# Autodesk Inventor assembly: MyPart_V0_with_case
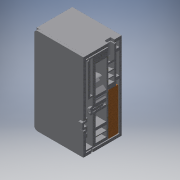
[picture p0: Inventor's stored thumbnail of the model, 180x180]
Saved by Autodesk Inventor 2016 (Build 200138000, 138)
## iProperties
Created: 2016-10-30
Part Number: MyPart_V0_with_case
Document SubType Name: Assembly
Designer: rawrdong
Author: rawrdong
## Documents named in this file (5)
- C:\Users\rawrdong\Box Sync\0_GradSchoolResearch\00_projects\0_AirParticleCounter\NEW_SHIT\MECH_E\MyPart_V0_with_case.iam
- C:\Users\rawrdong\Box Sync\0_GradSchoolResearch\00_projects\0_AirParticleCounter\NEW_SHIT\MECH_E\MyPart_V0.iam
- C:\Users\rawrdong\Box Sync\0_GradSchoolResearch\00_projects\0_AirParticleCounter\NEW_SHIT\MECH_E\case_button.ipt
- C:\Users\rawrdong\Box Sync\0_GradSchoolResearch\00_projects\0_AirParticleCounter\NEW_SHIT\MECH_E\case_carabiner.ipt
- C:\Users\rawrdong\Box Sync\0_GradSchoolResearch\00_projects\0_AirParticleCounter\NEW_SHIT\MECH_E\case_lid.ipt
## Components (4 placed, 4 different names)
1. MyPart_V0:1 [sub-assembly] — Mate:1, Flush:3, Flush:4, Flush:7, Flush:8
2. case_button:1 — Mate:3, Mate:4, Angle:1
3. case_carabiner:1 — Mate:1, Flush:1, Flush:2, Mate:2, Flush:5, Flush:6, Flush:9, Flush:10
4. case_lid:1 — Flush:1, Flush:2, Mate:2, Mate:3, Mate:4, Angle:1
## Relationships (21: Flush 10, Mate 6, Symmetry 4, Angle 1)
- Mate:1: MyPart_V0:1 ↔ case_carabiner:1
- Flush:1: case_carabiner:1 ↔ case_lid:1
- Flush:2: case_carabiner:1 ↔ case_lid:1
- Mate:2: case_carabiner:1 ↔ case_lid:1
- Mate:3: case_button:1 ↔ case_lid:1
- Mate:4: case_button:1 ↔ case_lid:1
- Angle:1 (180 deg): case_button:1 ↔ case_lid:1
- Flush:3: MyPart_V0:1
- Flush:4: MyPart_V0:1
- Symmetry:1
- Flush:5: case_carabiner:1
- Flush:6: case_carabiner:1
- Symmetry:2
- Mate:5
- Flush:7: MyPart_V0:1
- Flush:8: MyPart_V0:1
- Flush:9: case_carabiner:1
- Flush:10: case_carabiner:1
- Symmetry:3
- Symmetry:4
- Mate:6
